# Autodesk Inventor assembly: ICF34_ceramic_nipple_60mm
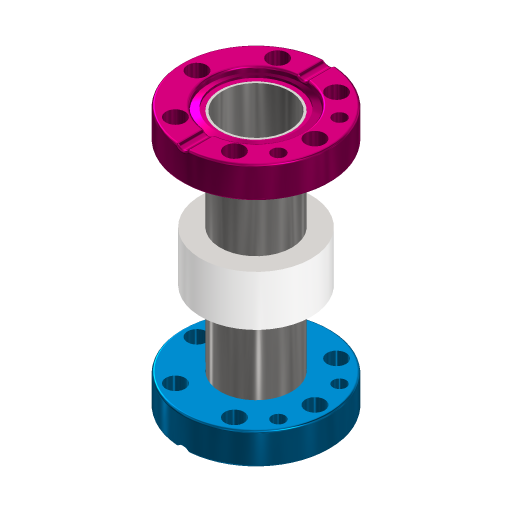
[picture p0: Inventor's stored thumbnail of the model, 512x512]
Saved by Autodesk Inventor 2024.2 (Build 282272000, 272)
## iProperties
Created: 2022-11-25
Part Number: ICF34_ceramic_nipple_60mm
Document SubType Name: Assembly
Designer: kuzmin
Author: kuzmin
## Documents named in this file (3)
- C:\Users\queez\Dropbox\Drawings\Leprecon\MovableProbe\ICF34_ceramic_nipple_60mm.iam
- C:\Users\queez\Dropbox\Drawings\Leprecon\MovableProbe\ICF34_Ceramic.ipt
- C:\Users\queez\Dropbox\Drawings\Leprecon\MovableProbe\cf34_ceramic_flange.ipt
## Components (3 placed, 2 different names)
1. ICF34_Ceramic:1 — Rotational:1, Rotational:2
2. cf34_ceramic_flange:1 — Rotational:1, Mate:1, Flush:1
3. cf34_ceramic_flange:2 — Rotational:2, Mate:1
## Relationships (4: RevoluteJoint 2, Mate 1, Flush 1)
- Rotational:1 [RevoluteJoint]: ICF34_Ceramic:1 ↔ cf34_ceramic_flange:1
- Rotational:2 [RevoluteJoint]: ICF34_Ceramic:1 ↔ cf34_ceramic_flange:2
- Mate:1: cf34_ceramic_flange:1 ↔ cf34_ceramic_flange:2
- Flush:1: cf34_ceramic_flange:1
